# Autodesk Inventor assembly: Day02_Task07
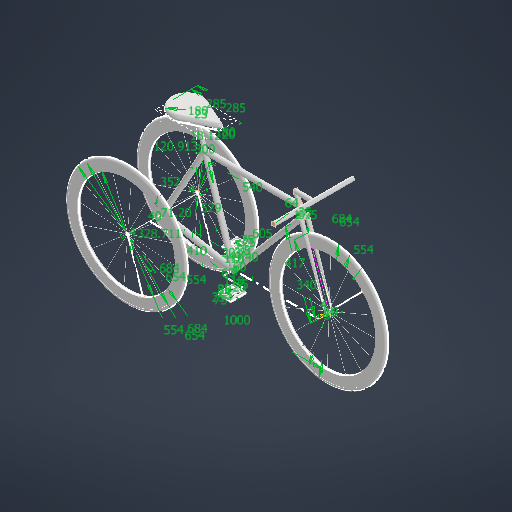
[picture p0: Inventor's stored thumbnail of the model, 512x512]
Saved by Autodesk Inventor 2026.3 (Build 303398000, 398)
## iProperties
Created: 2026-08-06
Part Number: Day02_Task07
Document SubType Name: Assembly
Designer: hojin
Author: hojin
## Documents named in this file (8)
- C:\robit_HW_design\day2\Day02_Task01_07\Day02_Task07\Day02_Task07.iam
- C:\robit_HW_design\day2\Day02_Task01_07\Day02_Task07\saddle.ipt
- C:\robit_HW_design\day2\Day02_Task01_07\Day02_Task07\wheel.ipt
- C:\robit_HW_design\day2\Day02_Task01_07\Day02_Task07\frame.ipt
- C:\robit_HW_design\day2\Day02_Task01_07\Day02_Task07\back_wheel_stick.ipt
- C:\robit_HW_design\day2\Day02_Task01_07\Day02_Task07\handle.ipt
- C:\robit_HW_design\day2\Day02_Task01_07\Day02_Task07\front_wheel_stick.ipt
- C:\robit_HW_design\day2\Day02_Task01_07\Day02_Task07\pedal.ipt
## Components (10 placed, 7 different names)
1. saddle:1 — 메이트:1, 각도:1, 회전:1, 메이트:2
2. wheel:1 — 강체:1
3. frame:1 — 메이트:1, 각도:1, 회전:1, 메이트:2, 강체:3, 메이트:3, 회전:1, 메이트:4
4. wheel:2 — 강체:2
5. wheel:3 — 회전:2
6. back_wheel_stick:1 — 강체:1, 강체:2, 강체:3
7. handle:1 — 메이트:3
8. front_wheel_stick:1 — 회전:1, 회전:2
9. pedal:2 — 회전:3
10. pedal:3 — 회전:3, 메이트:4
## Relationships (12: Mate 4, WeldJoint 3, RevoluteJoint 3, Angle 1, RelateRotation 1)
- 메이트:1 [Mate]: saddle:1 ↔ frame:1
- 각도:1 [Angle] (0 deg): saddle:1 ↔ frame:1
- 회전:1 [RelateRotation] (1 ul): saddle:1 ↔ frame:1
- 메이트:2 [Mate] (150 mm): saddle:1 ↔ frame:1
- 강체:1 [WeldJoint]: wheel:1 ↔ back_wheel_stick:1
- 강체:2 [WeldJoint]: wheel:2 ↔ back_wheel_stick:1
- 강체:3 [WeldJoint]: frame:1 ↔ back_wheel_stick:1
- 메이트:3 [Mate]: frame:1 ↔ handle:1
- 회전:1 [RevoluteJoint]: frame:1 ↔ front_wheel_stick:1
- 회전:2 [RevoluteJoint]: wheel:3 ↔ front_wheel_stick:1
- 회전:3 [RevoluteJoint]: pedal:2 ↔ pedal:3
- 메이트:4 [Mate]: frame:1 ↔ pedal:3
